# Autodesk Inventor assembly: CapBottomwChain
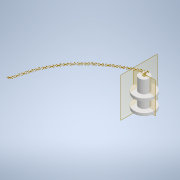
[picture p0: Inventor's stored thumbnail of the model, 180x180]
Saved by Autodesk Inventor 2021 (Build 250183000, 183)
## iProperties
Created: 2021-03-04
Part Number: CapBottomwChain
Document SubType Name: Assembly
Designer: CMurray
Author: CMurray
## Documents named in this file (3)
- F:\PHRC CADD 2021\2021 Game Design Challenge\Anchor\CapBottomwChain.iam
- F:\PHRC CADD 2021\2021 Game Design Challenge\Anchor\CapstanBottom-ver1-1111-2021.ipt
- F:\PHRC CADD 2021\2021 Game Design Challenge\Anchor\LongerChain.iam
## Components (2 placed, 2 different names)
1. CapstanBottom-ver1-1111-2021:1 — Mate:1
2. LongerChain:1 [sub-assembly] — Mate:1
## Relationships (1: Mate 1)
- Mate:1: CapstanBottom-ver1-1111-2021:1 ↔ LongerChain:1
